# Autodesk Inventor assembly: ElectronicLoad
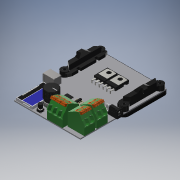
[picture p0: Inventor's stored thumbnail of the model, 180x180]
Saved by Autodesk Inventor 2018 (Build 220112000, 112)
## iProperties
Created: 2020-02-07
Part Number: ElectronicLoad
Document SubType Name: Assembly
Designer: Bradley
Author: Bradley
## Documents named in this file (14)
- C:\Users\Bradley\Documents\GitHub\CougsInSpace\Resources\Subsystems\Electronics\Testing\ElectronicLoad\CADModel\Native\ElectronicLoad.iam
- C:\Users\Bradley\Documents\GitHub\CougsInSpace\Resources\Subsystems\Electronics\Testing\ElectronicLoad\CADModel\Native\ElectronicLoad_PCB.ipt
- C:\Users\Bradley\Documents\GitHub\CougsInSpace\Resources\SupplierDocuments\05 - Connectors THT\05-0005\05-0005.ipt
- C:\Users\Bradley\Documents\GitHub\CougsInSpace\Resources\SupplierDocuments\05 - Connectors THT\05-0011\05-0011.ipt
- C:\Users\Bradley\Documents\GitHub\CougsInSpace\Resources\SupplierDocuments\05 - Connectors THT\05-0008\05-0008.ipt
- C:\Users\Bradley\Documents\GitHub\CougsInSpace\Resources\SupplierDocuments\05 - Connectors THT\05-0009\05-0009.ipt
- C:\Users\Bradley\Documents\GitHub\CougsInSpace\Resources\SupplierDocuments\04 - Connectors SMT\04-0004\04-0004.ipt
- C:\Users\Bradley\Documents\GitHub\CougsInSpace\Resources\SupplierDocuments\66 - Sensor\66-0006\66-0006.iam
- C:\Users\Bradley\Documents\GitHub\CougsInSpace\Resources\SupplierDocuments\03 - Board, Module, etc\03-0001\03-0001.ipt
- C:\Users\Bradley\Documents\GitHub\CougsInSpace\Resources\SupplierDocuments\05 - Connectors THT\05-0004\05-0004.ipt
- C:\Users\Bradley\Documents\GitHub\CougsInSpace\Resources\SupplierDocuments\61 - µController (and CLPD, FPGA,  etc.)\61-0002\61-0002.ipt
- C:\Users\Bradley\Documents\GitHub\CougsInSpace\Resources\SupplierDocuments\49 - Electromechanical\49-0005\49-0005.iam
- C:\Users\Bradley\Documents\GitHub\CougsInSpace\Resources\SupplierDocuments\48 - Hardware\48-0003\48-0003.iam
- C:\Users\Bradley\Documents\GitHub\CougsInSpace\Resources\SupplierDocuments\56 - Transistor FET\56-0008\56-0008-DOWN.ipt
## Components (15 placed, 13 different names)
1. ElectronicLoad_PCB:1 — Mate:1, Flush:1, Flush:2, Mate:2, Mate:3, Mate:4, Mate:5, Mate:6, Mate:7, Mate:8, Mate:9, Mate:10, Mate:11, Mate:12, Mate:13, Mate:14, Mate:15, Mate:16, Flush:5, Flush:6, Flush:7, Flush:8, Flush:9, Flush:10, Flush:11
2. 05-0005:1 — Mate:13, Flush:11
3. 05-0011:1 — Mate:12
4. 05-0008:1 — Mate:8, Flush:7, Mate:17
5. 05-0008:2 — Mate:9, Flush:5, Flush:6, Mate:17
6. 05-0009:1 — Mate:6, Flush:8, Flush:9
7. 04-0004:1 — Mate:14
8. 66-0006:1 [sub-assembly] — Mate:11
9. 03-0001:1 — Mate:7
10. 05-0004:1 — Mate:10, Flush:10
11. 61-0002:1 — Mate:15
12. 49-0005:1 [sub-assembly] — Mate:16
13. 48-0003:1 [sub-assembly] — Mate:1, Flush:1, Flush:2, Flush:3, Flush:4
14. 56-0008-DOWN:1 — Mate:3, Mate:4, Flush:4
15. 56-0008-DOWN:2 — Mate:2, Mate:5, Flush:3
## Relationships (28: Mate 17, Flush 11)
- Mate:1: ElectronicLoad_PCB:1 ↔ 48-0003:1
- Flush:1: ElectronicLoad_PCB:1 ↔ 48-0003:1
- Flush:2 (-32 mm): ElectronicLoad_PCB:1 ↔ 48-0003:1
- Mate:2 (1 mm): ElectronicLoad_PCB:1 ↔ 56-0008-DOWN:2
- Mate:3 (1 mm): ElectronicLoad_PCB:1 ↔ 56-0008-DOWN:1
- Mate:4 (8.5 mm): ElectronicLoad_PCB:1 ↔ 56-0008-DOWN:1
- Mate:5 (-8.5 mm): ElectronicLoad_PCB:1 ↔ 56-0008-DOWN:2
- Flush:3 (-1 mm): 48-0003:1 ↔ 56-0008-DOWN:2
- Flush:4 (-1 mm): 48-0003:1 ↔ 56-0008-DOWN:1
- Mate:6: ElectronicLoad_PCB:1 ↔ 05-0009:1
- Mate:7: ElectronicLoad_PCB:1 ↔ 03-0001:1
- Mate:8: ElectronicLoad_PCB:1 ↔ 05-0008:1
- Mate:9: ElectronicLoad_PCB:1 ↔ 05-0008:2
- Mate:10: ElectronicLoad_PCB:1 ↔ 05-0004:1
- Mate:11: ElectronicLoad_PCB:1 ↔ 66-0006:1
- Mate:12: ElectronicLoad_PCB:1 ↔ 05-0011:1
- Mate:13: ElectronicLoad_PCB:1 ↔ 05-0005:1
- Mate:14: ElectronicLoad_PCB:1 ↔ 04-0004:1
- Mate:15: ElectronicLoad_PCB:1 ↔ 61-0002:1
- Mate:16: ElectronicLoad_PCB:1 ↔ 49-0005:1
- Flush:5 (6 mm): ElectronicLoad_PCB:1 ↔ 05-0008:2
- Flush:6: ElectronicLoad_PCB:1 ↔ 05-0008:2
- Flush:7: ElectronicLoad_PCB:1 ↔ 05-0008:1
- Mate:17 (3 mm): 05-0008:1 ↔ 05-0008:2
- Flush:8: ElectronicLoad_PCB:1 ↔ 05-0009:1
- Flush:9 (27 mm): ElectronicLoad_PCB:1 ↔ 05-0009:1
- Flush:10 (-3 mm): ElectronicLoad_PCB:1 ↔ 05-0004:1
- Flush:11 (-3 mm): ElectronicLoad_PCB:1 ↔ 05-0005:1
